# Autodesk Inventor assembly: MotorAssembly
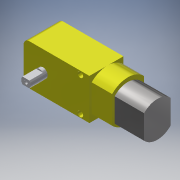
[picture p0: Inventor's stored thumbnail of the model, 180x180]
Saved by Autodesk Inventor 2018 (Build 220112000, 112)
## iProperties
Created: 2018-01-12
Part Number: MotorAssembly
Document SubType Name: Assembly
Designer: Kyle
Author: Kyle
## Documents named in this file (4)
- B:\My Documents\Project documentation\Hackathon-2018\Inventor\Robot\MotorAssembly.iam
- B:\My Documents\Project documentation\Hackathon-2018\Inventor\Robot\MotorFrame.ipt
- B:\My Documents\Project documentation\Hackathon-2018\Inventor\Robot\Motor.ipt
- B:\My Documents\Project documentation\Hackathon-2018\Inventor\Robot\MotorShaft.ipt
## Components (3 placed, 3 different names)
1. MotorFrame:1 — Mate:1, Mate:2, Angle:1, Mate:3, Mate:4, Mate:5
2. Motor:1 — Mate:1, Mate:2, Angle:1
3. MotorShaft:1 — Mate:3, Mate:4, Mate:5
## Relationships (6: Mate 5, Angle 1)
- Mate:1: MotorFrame:1 ↔ Motor:1
- Mate:2: MotorFrame:1 ↔ Motor:1
- Angle:1 (0 deg): MotorFrame:1 ↔ Motor:1
- Mate:3: MotorFrame:1 ↔ MotorShaft:1
- Mate:4 (-11.43 mm): MotorFrame:1 ↔ MotorShaft:1
- Mate:5 (-10.795 mm): MotorFrame:1 ↔ MotorShaft:1
